# Autodesk Inventor assembly: am-940a-6-HiGrip-_MIR1
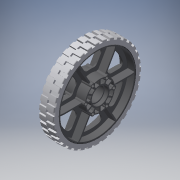
[picture p0: Inventor's stored thumbnail of the model, 180x180]
Saved by Autodesk Inventor 2017.3 (Build 213256000, 256)
## iProperties
Created: 2014-03-19
Part Number: am-940a-6-HiGrip-_MIR1
Description: STEP AP214
Document SubType Name: Assembly
Designer: steele
Sending System: SolidWorks 2010
Preprocessor: SwSTEP 2.0
Title: 6-HiGrip-am-940aSTEP.STEP
Revision Number: ANY
## Documents named in this file (3)
- D:\snobotics\CAD-Development\robSteele\SnoBotics2016\2016-01-23-BallShooter\am-940a-6-HiGrip-_MIR1.iam
- D:\snobotics\CAD-Development\robSteele\SnoBotics2016\2016-01-23-BallShooter\6 wheel Rev 4_MIR1.ipt
- D:\snobotics\CAD-Development\robSteele\SnoBotics2016\2016-01-23-BallShooter\6 wheel tread II_MIR1.ipt
## Components (2 placed, 2 different names)
1. 6 wheel Rev 4_MIR1:1
2. 6 wheel tread II_MIR1:1 — Flush:1
## Relationships (1: Flush 1)
- Flush:1 (-12.7 mm): 6 wheel tread II_MIR1:1
